# Autodesk Inventor assembly: Assembly_Cube_Kinematic_Mirrormount_Thorlabs_45_PRO_v3
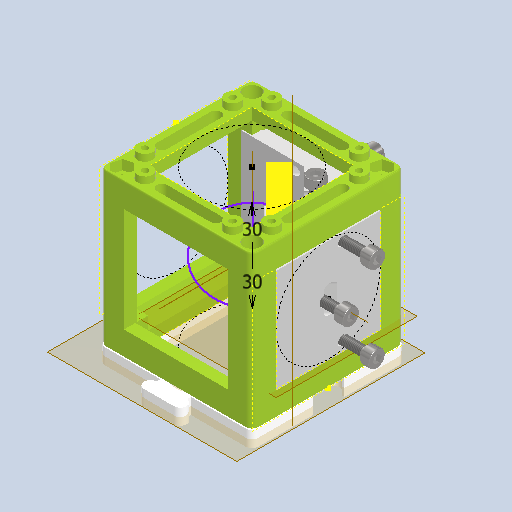
[picture p0: Inventor's stored thumbnail of the model, 512x512]
Saved by Autodesk Inventor 2022.3 (Build 263350000, 350)
## iProperties
Created: 2021-11-15
Part Number: Assembly_Cube_Kinematic_Mirrormount_Thorlabs_45_PRO_v3
Document SubType Name: Assembly
Designer: diederichbenedict
Author: diederichbenedict
## Documents named in this file (7)
- G:\My Drive\ASP - M.Sc. Photonics\Practical Modules\MODULE 4 - Master Thesis\2.Experiments\Modules\14.Mirror_45_Kinematic_Module\Kinematic_Mirror_Holder_45_edge\Assembly_Cube_Kinematic_Mirrormount_Thorlabs_45_PRO_v3.iam
- G:\My Drive\ASP - M.Sc. Photonics\Practical Modules\MODULE 4 - Master Thesis\2.Experiments\Modules\2.Base_Cube\Base_Cube_IM\Assembly_Cube_empty_IM_withBase_v3.iam
- G:\My Drive\ASP - M.Sc. Photonics\Practical Modules\MODULE 4 - Master Thesis\2.Experiments\Modules\14.Mirror_45_Kinematic_Module\Kinematic_Mirror_Holder_45_edge\00_Thorlabs_PF10-03-P01-Step.ipt
- G:\My Drive\ASP - M.Sc. Photonics\Practical Modules\MODULE 4 - Master Thesis\2.Experiments\Modules\14.Mirror_45_Kinematic_Module\Kinematic_Mirror_Holder_45_edge\20_Cube_Insert_Kinematic_KES400AMount_45_small_v3.ipt
- C:\Users\bingoeleda\Documents\Inventor\Content Center Files\R2022\en-US\DIN 912\DIN 912 - M3 x 0.5 x 12 x 10.75.ipt
- C:\Users\bingoeleda\Documents\Inventor\Content Center Files\R2022\en-US\DIN 912\DIN 912 - M3 x 0.5 x 16 x 14.75.ipt
- G:\My Drive\ASP - M.Sc. Photonics\Practical Modules\MODULE 4 - Master Thesis\2.Experiments\Modules\14.Mirror_45_Kinematic_Module\Kinematic_Mirror_Holder_45_edge\20_Cube_Insert_Kinematic_Mirror_45_pro_v3.ipt
## Components (9 placed, 6 different names)
1. 00_Thorlabs_PF10-03-P01-Step:1 — Rotational:1
2. 20_Cube_Insert_Kinematic_KES400AMount_45_small_v3:1 — Rigid:6, Rotational:1
3. Assembly_Cube_empty_IM_withBase_v3:1 [sub-assembly] — Mate:1, Flush:1, Mate:2, Flush:2, Flush:3
4. 20_Cube_Insert_Kinematic_Mirror_45_pro_v3:1 — Mate:1, Flush:1, Mate:2, Flush:2, Flush:3, Rigid:1, Rigid:2, Rigid:3, Rigid:4, Rigid:5, Rigid:6
5. DIN 912 - replaced by DIN EN ISO 4762 M3 x 16:1 — Rigid:3
6. DIN 912 - replaced by DIN EN ISO 4762 M3 x 16:2 — Rigid:5
7. DIN 912 - replaced by DIN EN ISO 4762 M3 x 12:3 — Rigid:2
8. DIN 912 - replaced by DIN EN ISO 4762 M3 x 12:4 — Rigid:1
9. DIN 912 - replaced by DIN EN ISO 4762 M3 x 16:3 — Rigid:4
## Relationships (12: WeldJoint 6, Flush 3, Mate 2, RevoluteJoint 1)
- Mate:1: Assembly_Cube_empty_IM_withBase_v3:1 ↔ 20_Cube_Insert_Kinematic_Mirror_45_pro_v3:1
- Flush:1: Assembly_Cube_empty_IM_withBase_v3:1 ↔ 20_Cube_Insert_Kinematic_Mirror_45_pro_v3:1
- Mate:2: Assembly_Cube_empty_IM_withBase_v3:1 ↔ 20_Cube_Insert_Kinematic_Mirror_45_pro_v3:1
- Flush:2: Assembly_Cube_empty_IM_withBase_v3:1 ↔ 20_Cube_Insert_Kinematic_Mirror_45_pro_v3:1
- Flush:3: Assembly_Cube_empty_IM_withBase_v3:1 ↔ 20_Cube_Insert_Kinematic_Mirror_45_pro_v3:1
- Rigid:1 [WeldJoint]: 20_Cube_Insert_Kinematic_Mirror_45_pro_v3:1 ↔ DIN 912 - replaced by DIN EN ISO 4762 M3 x 12:4
- Rigid:2 [WeldJoint]: 20_Cube_Insert_Kinematic_Mirror_45_pro_v3:1 ↔ DIN 912 - replaced by DIN EN ISO 4762 M3 x 12:3
- Rigid:3 [WeldJoint]: 20_Cube_Insert_Kinematic_Mirror_45_pro_v3:1 ↔ DIN 912 - replaced by DIN EN ISO 4762 M3 x 16:1
- Rigid:4 [WeldJoint]: 20_Cube_Insert_Kinematic_Mirror_45_pro_v3:1 ↔ DIN 912 - replaced by DIN EN ISO 4762 M3 x 16:3
- Rigid:5 [WeldJoint]: 20_Cube_Insert_Kinematic_Mirror_45_pro_v3:1 ↔ DIN 912 - replaced by DIN EN ISO 4762 M3 x 16:2
- Rigid:6 [WeldJoint]: 20_Cube_Insert_Kinematic_KES400AMount_45_small_v3:1 ↔ 20_Cube_Insert_Kinematic_Mirror_45_pro_v3:1
- Rotational:1 [RevoluteJoint]: 00_Thorlabs_PF10-03-P01-Step:1 ↔ 20_Cube_Insert_Kinematic_KES400AMount_45_small_v3:1
